# Autodesk Inventor assembly: shield
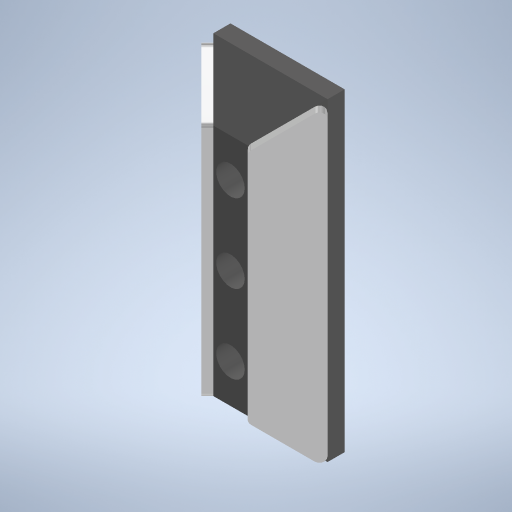
[picture p0: Inventor's stored thumbnail of the model, 512x512]
Saved by Autodesk Inventor 2024.1 (Build 281209000, 209)
## iProperties
Created: 2024-02-14
Part Number: shield
Document SubType Name: Assembly
Designer: hibik
Author: hibik
## Documents named in this file (3)
- C:\Users\hibik\Desktop\ロボメカ\HR\2024.02.11 Rl\02.11 ProtType\shield.iam
- C:\Users\hibik\Desktop\ロボメカ\HR\2024.02.11 Rl\02.11 ProtType\shield.ipt
- C:\Users\hibik\Desktop\ロボメカ\HR\2024.02.11 Rl\02.11 ProtType\shield_side_side.ipt
## Components (3 placed, 2 different names)
1. shield:1 — メイト:1, メイト:2, メイト:3, メイト:4, メイト:5, メイト:6
2. shield_side_side:1 — メイト:1, メイト:2, メイト:3
3. shield_side_side:2 — メイト:4, メイト:5, メイト:6
## Relationships (6: Mate 6)
- メイト:1 [Mate]: shield:1 ↔ shield_side_side:1
- メイト:2 [Mate]: shield:1 ↔ shield_side_side:1
- メイト:3 [Mate]: shield:1 ↔ shield_side_side:1
- メイト:4 [Mate]: shield:1 ↔ shield_side_side:2
- メイト:5 [Mate]: shield:1 ↔ shield_side_side:2
- メイト:6 [Mate]: shield:1 ↔ shield_side_side:2
